# Autodesk Inventor assembly: Lathe Model V3
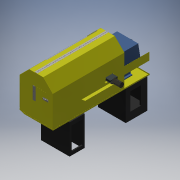
[picture p0: Inventor's stored thumbnail of the model, 180x180]
Saved by Autodesk Inventor 2018 (Build 220112000, 112)
## iProperties
Created: 2017-05-02
Part Number: Lathe Model V3
Document SubType Name: Assembly
Designer: M228544
Author: M228544
## Documents named in this file (46)
- C:\Users\P301319\Documents\GitHub\CNC-Lathe-CAD\CNC Lathe Project\Project Files\Lathe Model 2018.iam
- C:\Users\P301319\Documents\GitHub\CNC-Lathe-CAD\CNC Lathe Project\Project Files\BED.ipt
- C:\Users\P301319\Documents\GitHub\CNC-Lathe-CAD\CNC Lathe Project\Project Files\Bottom-Tool-Bit.ipt
- C:\Users\P301319\Documents\GitHub\CNC-Lathe-CAD\CNC Lathe Project\Project Files\Top-Part-Tool-bit.ipt
- C:\Users\P301319\Documents\GitHub\CNC-Lathe-CAD\CNC Lathe Project\Project Files\tail stock - body part.ipt
- C:\Users\P301319\Documents\GitHub\CNC-Lathe-CAD\CNC Lathe Project\Project Files\Left leg.ipt
- C:\Users\P301319\Documents\GitHub\CNC-Lathe-CAD\CNC Lathe Project\Project Files\Right Leg.ipt
- C:\Users\P301319\Documents\GitHub\CNC-Lathe-CAD\CNC Lathe Project\Project Files\Servo Motor\Servo Motor.iam
- C:\Users\P301319\Documents\GitHub\CNC-Lathe-CAD\CNC Lathe Project\Project Files\barrel.ipt
- C:\Users\P301319\Documents\GitHub\CNC-Lathe-CAD\CNC Lathe Project\Project Files\connecting wheel.ipt
- C:\Users\P301319\Documents\GitHub\CNC-Lathe-CAD\CNC Lathe Project\Project Files\chuck holder.ipt
- C:\Users\P301319\Documents\GitHub\CNC-Lathe-CAD\CNC Lathe Project\Project Files\Chuck shaft.ipt
- C:\Users\P301319\Documents\GitHub\CNC-Lathe-CAD\CNC Lathe Project\Project Files\X axis screw support.ipt
- C:\Users\P301319\Documents\GitHub\CNC-Lathe-CAD\CNC Lathe Project\Project Files\Assembly3.iam
- C:\Users\P301319\Documents\GitHub\CNC-Lathe-CAD\CNC Lathe Project\Project Files\Gearbox Handle.iam
- C:\Users\P301319\Documents\GitHub\CNC-Lathe-CAD\CNC Lathe Project\Project Files\Encoder Mount Hole Plug.ipt
- C:\Users\P301319\Documents\GitHub\CNC-Lathe-CAD\CNC Lathe Project\Project Files\Gearbox.ipt
- C:\Users\P301319\Documents\GitHub\CNC-Lathe-CAD\CNC Lathe Project\Project Files\Encoder Subassembly\Mounting.iam
- C:\Users\P301319\Documents\GitHub\CNC-Lathe-CAD\CNC Lathe Project\Project Files\X-axis Changes\slide-ontop-of-saddle.ipt
- C:\Users\P301319\Documents\GitHub\CNC-Lathe-CAD\CNC Lathe Project\Project Files\X-axis Changes\X Axis Shaft Assembly\short shaft x axis\shaft and nut.iam
- C:\Users\P301319\Documents\GitHub\CNC-Lathe-CAD\CNC Lathe Project\Project Files\X-axis Changes\Ball Screw\Correct nut unmodified ASSembly.iam
- C:\Users\P301319\Documents\GitHub\CNC-Lathe-CAD\CNC Lathe Project\Project Files\X-axis Changes\Ball Screw\X-axis Ball Screw Support.ipt
- C:\Users\P301319\Documents\GitHub\CNC-Lathe-CAD\CNC Lathe Project\Project Files\saddle.ipt
- C:\Users\P446024\Documents\GitHub\CNC-Lathe-CAD\CNC Lathe Project\Project Files\polycarbonate cover.ipt
- C:\Users\P301319\Documents\GitHub\CNC-Lathe-CAD\CNC Lathe Project\Project Files\Lathe Machine Cover parts 2018\cover\Part1.ipt
- C:\Users\P301319\Documents\GitHub\CNC-Lathe-CAD\CNC Lathe Project\Project Files\Lathe Machine Cover parts 2018\cover\Part2.ipt
- C:\Users\P301319\Documents\GitHub\CNC-Lathe-CAD\CNC Lathe Project\Project Files\Lathe Machine Cover parts 2018\cover\Cover V3\side plate.ipt
- C:\Users\P301319\Documents\GitHub\CNC-Lathe-CAD\CNC Lathe Project\Project Files\Updated Z axis\Z axis motor mount sub-assembly.iam
- C:\Users\P301319\Documents\GitHub\CNC-Lathe-CAD\CNC Lathe Project\Project Files\Lathe Machine Cover parts 2018\New Cover\Gearbox-Side Cover Part 1.ipt
- C:\Users\P301319\Documents\GitHub\CNC-Lathe-CAD\CNC Lathe Project\Project Files\Lathe Machine Cover parts 2018\New Cover\Gearbox-Side Cover Part 2.ipt
- C:\Users\P301319\Documents\GitHub\CNC-Lathe-CAD\CNC Lathe Project\Project Files\Lathe Machine Cover parts 2018\New Cover\Cover Lower Front.ipt
- C:\Users\P301319\Documents\GitHub\CNC-Lathe-CAD\CNC Lathe Project\Project Files\Lathe Machine Cover parts 2018\New Cover\NEW NEW COVER YAY\Back Panel.ipt
- C:\Users\P301319\Documents\GitHub\CNC-Lathe-CAD\CNC Lathe Project\Project Files\Lathe Machine Cover parts 2018\New Cover\NEW NEW COVER YAY\10mm Polycarb.ipt
- C:\Users\P301319\Documents\GitHub\CNC-Lathe-CAD\CNC Lathe Project\Project Files\Lathe Machine Cover parts 2018\New Cover\NEW NEW COVER YAY\Steel Front Door.ipt
- C:\Users\P301319\Documents\GitHub\CNC-Lathe-CAD\CNC Lathe Project\Project Files\Lathe Machine Cover parts 2018\New Cover\NEW NEW COVER YAY\Door.ipt
- C:\Users\P301319\Documents\GitHub\CNC-Lathe-CAD\CNC Lathe Project\Project Files\Lathe Machine Cover parts 2018\New Cover\NEW NEW COVER YAY\Little Hinge.ipt
- C:\Users\P301319\Documents\GitHub\CNC-Lathe-CAD\CNC Lathe Project\Project Files\Lathe Machine Cover parts 2018\New Cover\NEW NEW COVER YAY\Door Latch\Latch Base.ipt
- C:\Users\P301319\Documents\GitHub\CNC-Lathe-CAD\CNC Lathe Project\Project Files\Lathe Machine Cover parts 2018\New Cover\NEW NEW COVER YAY\Door Latch\Latch Catch.ipt
- C:\Users\P301319\Documents\GitHub\CNC-Lathe-CAD\CNC Lathe Project\Project Files\Lathe Machine Cover parts 2018\New Cover\NEW NEW COVER YAY\Door Latch\Latch Slide.ipt
- C:\Users\P301319\Documents\GitHub\CNC-Lathe-CAD\CNC Lathe Project\Project Files\Lathe Machine Cover parts 2018\New Cover\NEW NEW COVER YAY\Door Latch\Latch Catch Piece.ipt
- C:\Users\P301319\Documents\GitHub\CNC-Lathe-CAD\CNC Lathe Project\Project Files\Lathe Machine Cover parts 2018\New Cover\NEW NEW COVER YAY\X-Axis Panel Mount.ipt
- C:\Users\P301319\Documents\GitHub\CNC-Lathe-CAD\CNC Lathe Project\Project Files\Lathe Machine Cover parts 2018\New Cover\NEW NEW COVER YAY\X-Axis Panel Right.ipt
- C:\Users\P301319\Documents\GitHub\CNC-Lathe-CAD\CNC Lathe Project\Project Files\Lathe Machine Cover parts 2018\New Cover\NEW NEW COVER YAY\X-Axis Panel Left.ipt
- C:\Users\P301319\Documents\GitHub\CNC-Lathe-CAD\CNC Lathe Project\Project Files\Lathe Machine Cover parts 2018\New Cover\NEW NEW COVER YAY\Hinge 1 of 2.ipt
- C:\Users\P301319\Documents\GitHub\CNC-Lathe-CAD\CNC Lathe Project\Project Files\Lathe Machine Cover parts 2018\New Cover\NEW NEW COVER YAY\Hinge 2 of 2.ipt
- C:\Users\P301319\Documents\GitHub\CNC-Lathe-CAD\CNC Lathe Project\Project Files\Lathe Machine Cover parts 2018\New Cover\NEW NEW COVER YAY\Long Hinge.ipt
## Components (46 placed, 45 different names)
1. BED:1 — Mate:1, Mate:2, Mate:9, Mate:10, Mate:11, Flush:5, Flush:6, Mate:13, Mate:14, Flush:7, Flush:9, Flush:56, Mate:82, Mate:83, Mate:87
2. saddle:1 — Mate:1, Mate:2, Mate:5, Mate:6, Saddle and Slice on top of saddle, Mate:20, Flush:36, Angle:7, Mate:61, Mate:62
3. Bottom-Tool-Bit:1 — Mate:3, Mate:4, Flush:14
4. Top-Part-Tool-bit:1 — Mate:3, Mate:4, Mate:7, Mate:8, Tool Bit and Slece on top of saddle, Flush:14
5. slide-ontop-of-saddle:1 — Mate:5, Mate:6, Mate:7, Mate:8, Saddle and Slice on top of saddle, Tool Bit and Slece on top of saddle, Mate:70
6. tail stock - body part:1 — Mate:9, Mate:10, Flush:13, Mate:19, Mate:20, Mate:35, Mate:38, Flush:33
7. Gearbox:1 — Mate:11, Flush:5, Flush:13, Mate:19, Mate:39, Mate:40, Rotational:1, Mate:49, Flush:37, Mate:50, Mate:51, Mate:86, Mate:115
8. Left leg:1 — Mate:14, Flush:7, Flush:8, Mate:85
9. Right Leg:1 — Flush:6, Mate:13, Flush:8, Flush:9, Mate:130
10. barrel:1 — Mate:35, Mate:36, Mate:37, Rotation/Translation:1, Flush:33
11. connecting wheel:1 — Mate:36, Mate:37, Mate:38, Rotation/Translation:1
12. chuck holder:1 — Mate:39, Mate:40, Mate:41, Mate:42, Mate:48
13. Chuck shaft:1 — Mate:41, Mate:42, Mate:47
14. X axis screw support:1 — Flush:36, Mate:46, Mate:63, Mate:64, Angle:8, Mate:65, Mate:66, Mate:143, Mate:144, Mate:145
15. Servo Motor:2 [sub-assembly] — Mate:46, Angle:7, Mate:65, Mate:66
16. Assembly3:1 [sub-assembly] — Mate:47, Mate:48
17. Gearbox Handle:1 [sub-assembly] — Rotational:1
18. Encoder Mount Hole Plug:1 — Mate:49, Flush:37
19. Mounting:1 [sub-assembly] — Mate:50, Mate:51
20. shaft and nut:1 [sub-assembly] — Mate:61, Mate:62, Mate:63, Mate:64, Mate:67, Mate:69
21. Correct nut unmodified ASSembly:1 [sub-assembly] — Mate:67, Angle:9, Mate:68
22. X-axis Ball Screw Support:1 — Mate:68, Mate:69, Angle:10, Mate:70
23. polycarbonate cover:1
24. Part1:1
25. Part2:1
26. side plate:1 — Mate:127, Mate:128, Mate:129, Mate:131, Mate:139, Flush:79, Mate:140, Mate:157, Flush:82, Mate:159, Flush:83, Mate:160
27. Z axis motor mount sub-assembly:1 [sub-assembly] — Flush:56, Mate:82, Mate:83
28. Gearbox-Side Cover Part 1:1 — Mate:85, Mate:86, Mate:87, Mate:113, Mate:116, Flush:70, Mate:167
29. Gearbox-Side Cover Part 2:1 — Mate:115, Mate:116, Flush:70, Mate:118, Mate:119, Mate:121
30. Cover Lower Front:1 — Mate:113, Mate:130, Mate:131
31. Back Panel:1 — Mate:118, Mate:119, Mate:121, Mate:127, Mate:128, Mate:129, Mate:152, Mate:165, Flush:84
32. 10mm Polycarb:1 — Mate:124, Mate:125, Mate:126
33. Steel Front Door:1 — Mate:124, Mate:125, Mate:126, Mate:169, Mate:170, Flush:85
34. Door:1 — Mate:136, Flush:77, Flush:78, Mate:162, Mate:163, Mate:164
35. Latch Base:1 — Mate:136, Flush:77, Flush:78, Mate:137, Mate:138, Mate:142
36. Latch Catch:1 — Flush:80, Mate:141, Flush:81
37. Latch Slide:1 — Mate:137, Mate:138, Mate:142
38. Latch Catch Piece:1 — Mate:139, Flush:79, Mate:140, Flush:80, Mate:141, Flush:81
39. X-Axis Panel Mount:1 — Mate:143, Mate:144, Mate:145, Mate:146, Mate:147, Mate:148, Mate:152, Mate:153, Mate:154, Mate:155
40. X-Axis Panel Right:1 — Mate:146, Mate:147, Mate:148
41. X-Axis Panel Left:1 — Mate:153, Mate:154, Mate:155
42. Hinge 1 of 2:1 — Mate:158, Rotational:3, Mate:162, Mate:163, Mate:164
43. Hinge 2 of 2:1 — Mate:157, Flush:82, Mate:158, Rotational:3, Mate:161
44. Little Hinge:1 — Mate:159, Flush:83, Mate:160, Mate:161
45. Long Hinge:1 — Mate:168, Rotational:4, Mate:169, Mate:170, Flush:85
46. Long Hinge:2 — Mate:165, Mate:167, Mate:168, Rotational:4, Flush:84
## Relationships (119: Mate 88, Flush 22, Angle 5, RevoluteJoint 3, RelateRotateTranslate 1)
- Mate:1: BED:1 ↔ saddle:1
- Mate:2: BED:1 ↔ saddle:1
- Mate:3: Bottom-Tool-Bit:1 ↔ Top-Part-Tool-bit:1
- Mate:4: Bottom-Tool-Bit:1 ↔ Top-Part-Tool-bit:1
- Mate:5: saddle:1 ↔ slide-ontop-of-saddle:1
- Mate:6: saddle:1 ↔ slide-ontop-of-saddle:1
- Mate:7: Top-Part-Tool-bit:1 ↔ slide-ontop-of-saddle:1
- Mate:8: Top-Part-Tool-bit:1 ↔ slide-ontop-of-saddle:1
- Mate:9: BED:1 ↔ tail stock - body part:1
- Mate:10: BED:1 ↔ tail stock - body part:1
- Saddle and Slice on top of saddle [Flush]: saddle:1 ↔ slide-ontop-of-saddle:1
- Tool Bit and Slece on top of saddle [Angle] (-90 deg): Top-Part-Tool-bit:1 ↔ slide-ontop-of-saddle:1
- Mate:11: BED:1 ↔ Gearbox:1
- Flush:5: BED:1 ↔ Gearbox:1
- Flush:13: tail stock - body part:1 ↔ Gearbox:1
- Flush:6: BED:1 ↔ Right Leg:1
- Mate:13: BED:1 ↔ Right Leg:1
- Mate:14: BED:1 ↔ Left leg:1
- Flush:7: BED:1 ↔ Left leg:1
- Flush:8: Left leg:1 ↔ Right Leg:1
- Flush:9 (145 mm): BED:1 ↔ Right Leg:1
- Flush:14: Bottom-Tool-Bit:1 ↔ Top-Part-Tool-bit:1
- Mate:19: tail stock - body part:1 ↔ Gearbox:1
- Mate:20: saddle:1 ↔ tail stock - body part:1
- Mate:35: tail stock - body part:1 ↔ barrel:1
- Mate:36: barrel:1 ↔ connecting wheel:1
- Mate:37: barrel:1 ↔ connecting wheel:1
- Mate:38: tail stock - body part:1 ↔ connecting wheel:1
- Rotation/Translation:1 [RelateRotateTranslate] (100 mm): barrel:1 ↔ connecting wheel:1
- Flush:33: tail stock - body part:1 ↔ barrel:1
- Mate:39: Gearbox:1 ↔ chuck holder:1
- Mate:40 (0.46 mm): Gearbox:1 ↔ chuck holder:1
- Mate:41: chuck holder:1 ↔ Chuck shaft:1
- Mate:42 (11.2 mm): chuck holder:1 ↔ Chuck shaft:1
- Flush:36: saddle:1 ↔ X axis screw support:1
- Mate:46: X axis screw support:1 ↔ Servo Motor:2
- Angle:7 (225 deg): saddle:1 ↔ Servo Motor:2
- Mate:47: Chuck shaft:1 ↔ Assembly3:1
- Mate:48: chuck holder:1 ↔ Assembly3:1
- Rotational:1 [RevoluteJoint]: Gearbox:1 ↔ Gearbox Handle:1
- Mate:49: Gearbox:1 ↔ Encoder Mount Hole Plug:1
- Flush:37: Gearbox:1 ↔ Encoder Mount Hole Plug:1
- Mate:50: Gearbox:1 ↔ Mounting:1
- Mate:51: Gearbox:1 ↔ Mounting:1
- Mate:61: saddle:1 ↔ shaft and nut:1
- Mate:62: saddle:1 ↔ shaft and nut:1
- Mate:63: X axis screw support:1 ↔ shaft and nut:1
- Mate:64 (-50 mm): X axis screw support:1 ↔ shaft and nut:1
- Angle:8 (180 deg): X axis screw support:1
- Mate:65: X axis screw support:1 ↔ Servo Motor:2
- Mate:66: X axis screw support:1 ↔ Servo Motor:2
- Mate:67: shaft and nut:1 ↔ Correct nut unmodified ASSembly:1
- Angle:9 (180 deg): Correct nut unmodified ASSembly:1
- Mate:68: Correct nut unmodified ASSembly:1 ↔ X-axis Ball Screw Support:1
- Mate:69: shaft and nut:1 ↔ X-axis Ball Screw Support:1
- Angle:10 (90 deg): X-axis Ball Screw Support:1
- Mate:70 (-261 mm): slide-ontop-of-saddle:1 ↔ X-axis Ball Screw Support:1
- Flush:56: BED:1 ↔ Z axis motor mount sub-assembly:1
- Mate:82: BED:1 ↔ Z axis motor mount sub-assembly:1
- Mate:83: BED:1 ↔ Z axis motor mount sub-assembly:1
- Mate:85 (15 mm): Left leg:1 ↔ Gearbox-Side Cover Part 1:1
- Mate:86: Gearbox:1 ↔ Gearbox-Side Cover Part 1:1
- Mate:87: BED:1 ↔ Gearbox-Side Cover Part 1:1
- Mate:113: Gearbox-Side Cover Part 1:1 ↔ Cover Lower Front:1
- Mate:115: Gearbox:1 ↔ Gearbox-Side Cover Part 2:1
- Mate:116: Gearbox-Side Cover Part 1:1 ↔ Gearbox-Side Cover Part 2:1
- Flush:70: Gearbox-Side Cover Part 1:1 ↔ Gearbox-Side Cover Part 2:1
- Mate:118: Gearbox-Side Cover Part 2:1 ↔ Back Panel:1
- Mate:119: Gearbox-Side Cover Part 2:1 ↔ Back Panel:1
- Mate:121: Gearbox-Side Cover Part 2:1 ↔ Back Panel:1
- Mate:124: 10mm Polycarb:1 ↔ Steel Front Door:1
- Mate:125: 10mm Polycarb:1 ↔ Steel Front Door:1
- Mate:126 (-50 mm): 10mm Polycarb:1 ↔ Steel Front Door:1
- Mate:127: side plate:1 ↔ Back Panel:1
- Mate:128: side plate:1 ↔ Back Panel:1
- Mate:129: side plate:1 ↔ Back Panel:1
- Mate:130: Right Leg:1 ↔ Cover Lower Front:1
- Mate:131: side plate:1 ↔ Cover Lower Front:1
- Mate:136: Door:1 ↔ Latch Base:1
- Flush:77: Door:1 ↔ Latch Base:1
- Flush:78 (100 mm): Door:1 ↔ Latch Base:1
- Mate:137: Latch Base:1 ↔ Latch Slide:1
- Mate:138: Latch Base:1 ↔ Latch Slide:1
- Mate:139: side plate:1 ↔ Latch Catch Piece:1
- Flush:79 (17.5 mm): side plate:1 ↔ Latch Catch Piece:1
- Mate:140 (85 mm): side plate:1 ↔ Latch Catch Piece:1
- Flush:80: Latch Catch:1 ↔ Latch Catch Piece:1
- Mate:141: Latch Catch:1 ↔ Latch Catch Piece:1
- Flush:81: Latch Catch:1 ↔ Latch Catch Piece:1
- Mate:142: Latch Base:1 ↔ Latch Slide:1
- Mate:143: X axis screw support:1 ↔ X-Axis Panel Mount:1
- Mate:144: X axis screw support:1 ↔ X-Axis Panel Mount:1
- Mate:145: X axis screw support:1 ↔ X-Axis Panel Mount:1
- Mate:146: X-Axis Panel Mount:1 ↔ X-Axis Panel Right:1
- Mate:147: X-Axis Panel Mount:1 ↔ X-Axis Panel Right:1
- Mate:148: X-Axis Panel Mount:1 ↔ X-Axis Panel Right:1
- Mate:152: Back Panel:1 ↔ X-Axis Panel Mount:1
- Mate:153: X-Axis Panel Mount:1 ↔ X-Axis Panel Left:1
- Mate:154: X-Axis Panel Mount:1 ↔ X-Axis Panel Left:1
- Mate:155: X-Axis Panel Mount:1 ↔ X-Axis Panel Left:1
- Mate:157 (-15 mm): side plate:1 ↔ Hinge 2 of 2:1
- Flush:82 (20 mm): side plate:1 ↔ Hinge 2 of 2:1
- Mate:158: Hinge 1 of 2:1 ↔ Hinge 2 of 2:1
- Rotational:3 [RevoluteJoint]: Hinge 1 of 2:1 ↔ Hinge 2 of 2:1
- Mate:159: side plate:1 ↔ Little Hinge:1
- Flush:83 (20 mm): side plate:1 ↔ Little Hinge:1
- Mate:160 (-15 mm): side plate:1 ↔ Little Hinge:1
- Mate:161: Hinge 2 of 2:1 ↔ Little Hinge:1
- Mate:162: Door:1 ↔ Hinge 1 of 2:1
- Mate:163: Door:1 ↔ Hinge 1 of 2:1
- Mate:164: Door:1 ↔ Hinge 1 of 2:1
- Mate:165: Back Panel:1 ↔ Long Hinge:2
- Mate:167 (1.8 mm): Gearbox-Side Cover Part 1:1 ↔ Long Hinge:2
- Mate:168: Long Hinge:1 ↔ Long Hinge:2
- Rotational:4 [RevoluteJoint]: Long Hinge:1 ↔ Long Hinge:2
- Mate:169: Steel Front Door:1 ↔ Long Hinge:1
- Mate:170 (1.8 mm): Steel Front Door:1 ↔ Long Hinge:1
- Flush:84: Back Panel:1 ↔ Long Hinge:2
- Flush:85: Steel Front Door:1 ↔ Long Hinge:1
